# Autodesk Inventor assembly: Dai
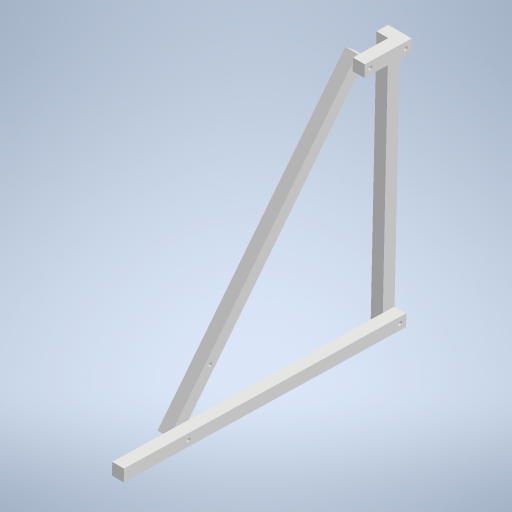
[picture p0: Inventor's stored thumbnail of the model, 512x512]
Saved by Autodesk Inventor 2023 (Build 270158000, 158)
## iProperties
Created: 2022-10-24
Part Number: Dai
Document SubType Name: Assembly
Designer: banru
Author: banru
## Documents named in this file (5)
- C:\Users\banru\Documents\workspace\Contactless\Inventor\Dai\Dai.iam
- C:\Users\banru\Documents\workspace\Contactless\Inventor\Dai\Dai.ipt
- C:\Users\banru\Documents\workspace\Contactless\Inventor\Dai\Naname.ipt
- C:\Users\banru\Documents\workspace\Contactless\Inventor\Dai\Tate.ipt
- C:\Users\banru\Documents\workspace\Contactless\Inventor\Dai\DaiUe.ipt
## Components (4 placed, 4 different names)
1. Dai:1 — 挿入:1, 挿入:2, フラッシュ:1
2. Naname:1 — 挿入:2, 挿入:4
3. Tate:1 — 挿入:1, 挿入:3, フラッシュ:1
4. DaiUe:1 — 挿入:3, 挿入:4
## Relationships (5: Insert 4, Flush 1)
- 挿入:1 [Insert]: Dai:1 ↔ Tate:1
- 挿入:2 [Insert]: Dai:1 ↔ Naname:1
- 挿入:3 [Insert]: Tate:1 ↔ DaiUe:1
- 挿入:4 [Insert]: Naname:1 ↔ DaiUe:1
- フラッシュ:1 [Flush]: Dai:1 ↔ Tate:1
